# Autodesk Inventor assembly: khung
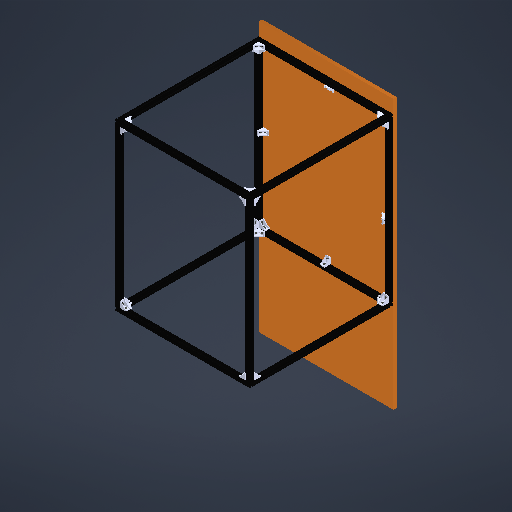
[picture p0: Inventor's stored thumbnail of the model, 512x512]
Saved by Autodesk Inventor 2027.1 (Build 311270010, 270A)
## iProperties
Created: 2026-08-09
Part Number: khung
Document SubType Name: Assembly
Designer: MSI
Author: MSI
## Documents named in this file (6)
- C:\Users\MSI\Documents\MECHATRONICS\Tot_nghiep\Do_an_Delta.Robot_Dang_Rui_Bi\Thiết kế\Delta Part\khung.iam
- C:\Users\MSI\Documents\MECHATRONICS\Tot_nghiep\Do_an_Delta.Robot_Dang_Rui_Bi\Thiết kế\Delta Part\tấm gỗ.ipt
- C:\Users\MSI\Documents\MECHATRONICS\Tot_nghiep\Do_an_Delta.Robot_Dang_Rui_Bi\Thiết kế\Delta Part\nhôm định hình 20x20_600.ipt
- C:\Users\MSI\Documents\MECHATRONICS\Tot_nghiep\Do_an_Delta.Robot_Dang_Rui_Bi\Thiết kế\Delta Part\nhôm định hình 20x20_700.ipt
- C:\Users\MSI\Documents\MECHATRONICS\Tot_nghiep\Do_an_Delta.Robot_Dang_Rui_Bi\Thiết kế\Delta Part\ke góc.ipt
- C:\Users\MSI\Documents\Inventor\Content Center Files\R2027\en-US\ISO 7380-1\ISO 7380-1 - M5 x 8.ipt
## Components (100 placed, 5 different names)
1. tấm gỗ:1 — Flush:1, Mate:1, Flush:2, Mate:3, Flush:4, Mate:5, Flush:5, Mate:66, Mate:67, Mate:68, Mate:69
2. nhôm định hình 20x20_600:1 — Flush:1, Mate:1, Mate:2, Flush:3, Mate:4, Mate:10, Flush:10, Flush:11, Mate:11, Flush:12, Flush:13, Mate:21, Mate:22, Flush:24, Mate:27, Mate:30, Flush:28, Mate:71
3. nhôm định hình 20x20_700:1 — Mate:2, Flush:2, Flush:3, Mate:7, Mate:19, Mate:20, Flush:22, Flush:23, Mate:32, Flush:29, Mate:36, Mate:70
4. nhôm định hình 20x20_700:2 — Mate:3, Flush:4, Mate:4, Mate:6, Mate:8, Flush:6, Mate:23, Mate:25, Mate:28, Mate:38, Mate:73
5. nhôm định hình 20x20_600:2 — Mate:5, Mate:6, Mate:7, Flush:5, Flush:7, Mate:9, Flush:8, Flush:9, Mate:18, Mate:24, Flush:25, Mate:35, Mate:40, Mate:72
6. nhôm định hình 20x20_600:3 — Mate:10, Flush:10, Flush:11, Mate:13, Mate:31, Mate:33, Mate:54, Mate:56, Flush:41
7. nhôm định hình 20x20_600:4 — Mate:11, Flush:12, Flush:13, Mate:12, Flush:14, Flush:15, Mate:14, Mate:26, Flush:26, Mate:29, Flush:27, Mate:50, Mate:52
8. nhôm định hình 20x20_600:5 — Mate:9, Flush:8, Flush:9, Mate:15, Flush:17, Mate:34, Flush:30, Mate:37, Flush:31, Mate:43, Flush:34, Mate:44
9. nhôm định hình 20x20_600:6 — Mate:8, Flush:6, Flush:7, Flush:16, Mate:39, Flush:32, Mate:41, Flush:33, Mate:46, Flush:36, Mate:48
10. nhôm định hình 20x20_600:7 — Mate:15, Flush:16, Flush:17, Mate:16, Flush:19, Mate:17, Mate:42, Mate:47, Mate:59, Flush:42, Mate:64, Flush:45
11. nhôm định hình 20x20_600:8 — Mate:12, Mate:13, Flush:14, Flush:15, Mate:14, Flush:18, Flush:20, Flush:21, Mate:53, Flush:39, Mate:55, Flush:40, Mate:61, Flush:43, Mate:62
12. nhôm định hình 20x20_700:3 — Mate:16, Flush:18, Flush:19, Mate:45, Flush:35, Mate:57, Mate:58, Mate:60
13. nhôm định hình 20x20_700:4 — Mate:17, Flush:20, Flush:21, Mate:49, Flush:37, Mate:51, Flush:38, Mate:63, Flush:44, Mate:65
14. ke góc:1 — Mate:28, Mate:29, Flush:27, Insert:23, Insert:24
15. ke góc:2 — Mate:32, Mate:33, Flush:29, Insert:31, Insert:32
16. ke góc:3 — Mate:38, Mate:39, Flush:32, Insert:5, Insert:6, Insert:9
17. ke góc:4 — Mate:36, Mate:37, Flush:31, Insert:12, Insert:13
18. ke góc:5 — Mate:34, Mate:35, Flush:30, Insert:16, Insert:17
19. ke góc:6 — Mate:26, Mate:27, Flush:26, Insert:21, Insert:22
20. ke góc:7 — Mate:24, Mate:25, Flush:25, Insert:1, Insert:2, Insert:3, Insert:4
21. ke góc:8 — Mate:18, Mate:19, Flush:23, Insert:14, Insert:15
22. ke góc:9 — Mate:22, Flush:24, Mate:23, Insert:25, Insert:26
23. ke góc:10 — Mate:20, Mate:21, Flush:22, Insert:29, Insert:30
24. ke góc:11 — Mate:30, Mate:31, Flush:28, Insert:33, Insert:34
25. ke góc:12 — Mate:46, Mate:47, Flush:36, Insert:39, Insert:40
26. ke góc:13 — Mate:58, Mate:59, Flush:42, Insert:54, Insert:55
27. ke góc:14 — Mate:56, Mate:57, Flush:41, Insert:47, Insert:52
28. ke góc:15 — Mate:52, Mate:53, Flush:39, Insert:41, Insert:42
29. ke góc:16 — Mate:48, Mate:49, Flush:37, Insert:35, Insert:37
30. ke góc:17 — Mate:50, Mate:51, Flush:38, Insert:45, Insert:46
31. ke góc:18 — Mate:44, Mate:45, Flush:35, Insert:57, Insert:58
32. ke góc:19 — Mate:42, Mate:43, Flush:34, Insert:53, Insert:56
33. ke góc:20 — Mate:54, Mate:55, Flush:40, Insert:50, Insert:51
34. ke góc:21 — Mate:40, Mate:41, Flush:33, Insert:7, Insert:8
35. ke góc:22 — Mate:60, Mate:61, Flush:43, Insert:48, Insert:49
36. ke góc:23 — Mate:62, Mate:63, Flush:44, Insert:43, Insert:44
37. ke góc:24 — Mate:64, Mate:65, Flush:45, Insert:36, Insert:38
38. ke góc:25 — Mate:66, Mate:70, Mate:74, Mate:75, Insert:18
39. ke góc:26 — Mate:69, Mate:72, Insert:10, Insert:11
40. ke góc:27 — Mate:68, Mate:71, Insert:27, Insert:28
41. ke góc:28 — Mate:67, Mate:73, Insert:19, Insert:20
42. ISO 7380-1 M5 x 8:1 — Insert:1
43. ISO 7380-1 M5 x 8:2 — Insert:2
44. ISO 7380-1 M5 x 8:3 — Insert:3
45. ISO 7380-1 M5 x 8:4 — Insert:4
46. ISO 7380-1 M5 x 8:5 — Insert:5
47. ISO 7380-1 M5 x 8:6 — Insert:6
48. ISO 7380-1 M5 x 8:7 — Insert:7
49. ISO 7380-1 M5 x 8:8 — Insert:8
50. ISO 7380-1 M5 x 8:9 — Insert:9
51. ISO 7380-1 M5 x 8:10 — Insert:10
52. ISO 7380-1 M5 x 8:11 — Insert:11
53. ISO 7380-1 M5 x 8:12 — Insert:12
54. ISO 7380-1 M5 x 8:13 — Insert:13
55. ISO 7380-1 M5 x 8:14 — Insert:14
56. ISO 7380-1 M5 x 8:15 — Insert:15
57. ISO 7380-1 M5 x 8:16 — Insert:16
58. ISO 7380-1 M5 x 8:17 — Insert:17
59. ISO 7380-1 M5 x 8:18 — Mate:74, Mate:75
60. ISO 7380-1 M5 x 8:19 — Insert:18
61. ISO 7380-1 M5 x 8:20 — Insert:19
62. ISO 7380-1 M5 x 8:21 — Insert:20
63. ISO 7380-1 M5 x 8:22 — Insert:21
64. ISO 7380-1 M5 x 8:23 — Insert:22
65. ISO 7380-1 M5 x 8:24 — Insert:23
66. ISO 7380-1 M5 x 8:25 — Insert:24
67. ISO 7380-1 M5 x 8:26 — Insert:25
68. ISO 7380-1 M5 x 8:27 — Insert:26
69. ISO 7380-1 M5 x 8:28 — Insert:27
70. ISO 7380-1 M5 x 8:29 — Insert:28
71. ISO 7380-1 M5 x 8:30 — Insert:29
72. ISO 7380-1 M5 x 8:31 — Insert:30
73. ISO 7380-1 M5 x 8:32 — Insert:31
74. ISO 7380-1 M5 x 8:33 — Insert:32
75. ISO 7380-1 M5 x 8:34 — Insert:33
76. ISO 7380-1 M5 x 8:35 — Insert:34
77. ISO 7380-1 M5 x 8:36 — Insert:35
78. ISO 7380-1 M5 x 8:37 — Insert:36
79. ISO 7380-1 M5 x 8:38 — Insert:37
80. ISO 7380-1 M5 x 8:39 — Insert:38
81. ISO 7380-1 M5 x 8:40 — Insert:39
82. ISO 7380-1 M5 x 8:41 — Insert:40
83. ISO 7380-1 M5 x 8:42 — Insert:41
84. ISO 7380-1 M5 x 8:43 — Insert:42
85. ISO 7380-1 M5 x 8:44 — Insert:43
86. ISO 7380-1 M5 x 8:45 — Insert:44
87. ISO 7380-1 M5 x 8:46 — Insert:45
88. ISO 7380-1 M5 x 8:47 — Insert:46
89. ISO 7380-1 M5 x 8:48 — Insert:47
90. ISO 7380-1 M5 x 8:49 — Insert:48
91. ISO 7380-1 M5 x 8:50 — Insert:49
92. ISO 7380-1 M5 x 8:51 — Insert:50
93. ISO 7380-1 M5 x 8:52 — Insert:51
94. ISO 7380-1 M5 x 8:53 — Insert:52
95. ISO 7380-1 M5 x 8:54 — Insert:53
96. ISO 7380-1 M5 x 8:55 — Insert:54
97. ISO 7380-1 M5 x 8:56 — Insert:55
98. ISO 7380-1 M5 x 8:57 — Insert:56
99. ISO 7380-1 M5 x 8:58 — Insert:57
100. ISO 7380-1 M5 x 8:59 — Insert:58
## Relationships (178: Mate 75, Insert 58, Flush 45)
- Flush:1: tấm gỗ:1 ↔ nhôm định hình 20x20_600:1
- Mate:1: tấm gỗ:1 ↔ nhôm định hình 20x20_600:1
- Mate:2: nhôm định hình 20x20_600:1 ↔ nhôm định hình 20x20_700:1
- Flush:2: tấm gỗ:1 ↔ nhôm định hình 20x20_700:1
- Flush:3: nhôm định hình 20x20_600:1 ↔ nhôm định hình 20x20_700:1
- Mate:3: tấm gỗ:1 ↔ nhôm định hình 20x20_700:2
- Flush:4: tấm gỗ:1 ↔ nhôm định hình 20x20_700:2
- Mate:4: nhôm định hình 20x20_600:1 ↔ nhôm định hình 20x20_700:2
- Mate:5: tấm gỗ:1 ↔ nhôm định hình 20x20_600:2
- Mate:6: nhôm định hình 20x20_700:2 ↔ nhôm định hình 20x20_600:2
- Mate:7: nhôm định hình 20x20_700:1 ↔ nhôm định hình 20x20_600:2
- Flush:5: tấm gỗ:1 ↔ nhôm định hình 20x20_600:2
- Mate:8: nhôm định hình 20x20_700:2 ↔ nhôm định hình 20x20_600:6
- Flush:6: nhôm định hình 20x20_700:2 ↔ nhôm định hình 20x20_600:6
- Flush:7: nhôm định hình 20x20_600:2 ↔ nhôm định hình 20x20_600:6
- Mate:9: nhôm định hình 20x20_600:2 ↔ nhôm định hình 20x20_600:5
- Flush:8: nhôm định hình 20x20_600:2 ↔ nhôm định hình 20x20_600:5
- Flush:9: nhôm định hình 20x20_600:2 ↔ nhôm định hình 20x20_600:5
- Mate:10: nhôm định hình 20x20_600:1 ↔ nhôm định hình 20x20_600:3
- Flush:10: nhôm định hình 20x20_600:1 ↔ nhôm định hình 20x20_600:3
- Flush:11: nhôm định hình 20x20_600:1 ↔ nhôm định hình 20x20_600:3
- Mate:11: nhôm định hình 20x20_600:1 ↔ nhôm định hình 20x20_600:4
- Flush:12: nhôm định hình 20x20_600:1 ↔ nhôm định hình 20x20_600:4
- Flush:13: nhôm định hình 20x20_600:1 ↔ nhôm định hình 20x20_600:4
- Mate:12: nhôm định hình 20x20_600:4 ↔ nhôm định hình 20x20_600:8
- Mate:13: nhôm định hình 20x20_600:3 ↔ nhôm định hình 20x20_600:8
- Flush:14: nhôm định hình 20x20_600:4 ↔ nhôm định hình 20x20_600:8
- Flush:15: nhôm định hình 20x20_600:4 ↔ nhôm định hình 20x20_600:8
- Mate:14: nhôm định hình 20x20_600:4 ↔ nhôm định hình 20x20_600:8
- Mate:15: nhôm định hình 20x20_600:5 ↔ nhôm định hình 20x20_600:7
- Flush:16: nhôm định hình 20x20_600:6 ↔ nhôm định hình 20x20_600:7
- Flush:17: nhôm định hình 20x20_600:5 ↔ nhôm định hình 20x20_600:7
- Mate:16: nhôm định hình 20x20_600:7 ↔ nhôm định hình 20x20_700:3
- Flush:18: nhôm định hình 20x20_600:8 ↔ nhôm định hình 20x20_700:3
- Flush:19: nhôm định hình 20x20_600:7 ↔ nhôm định hình 20x20_700:3
- Mate:17: nhôm định hình 20x20_600:7 ↔ nhôm định hình 20x20_700:4
- Flush:20: nhôm định hình 20x20_600:8 ↔ nhôm định hình 20x20_700:4
- Flush:21: nhôm định hình 20x20_600:8 ↔ nhôm định hình 20x20_700:4
- Mate:18: nhôm định hình 20x20_600:2 ↔ ke góc:8
- Mate:19: nhôm định hình 20x20_700:1 ↔ ke góc:8
- Mate:20: nhôm định hình 20x20_700:1 ↔ ke góc:10
- Mate:21: nhôm định hình 20x20_600:1 ↔ ke góc:10
- Flush:22: nhôm định hình 20x20_700:1 ↔ ke góc:10
- Flush:23: nhôm định hình 20x20_700:1 ↔ ke góc:8
- Mate:22: nhôm định hình 20x20_600:1 ↔ ke góc:9
- Flush:24: nhôm định hình 20x20_600:1 ↔ ke góc:9
- Mate:23: nhôm định hình 20x20_700:2 ↔ ke góc:9
- Mate:24: nhôm định hình 20x20_600:2 ↔ ke góc:7
- Mate:25: nhôm định hình 20x20_700:2 ↔ ke góc:7
- Flush:25: nhôm định hình 20x20_600:2 ↔ ke góc:7
- Mate:26: nhôm định hình 20x20_600:4 ↔ ke góc:6
- Mate:27: nhôm định hình 20x20_600:1 ↔ ke góc:6
- Flush:26: nhôm định hình 20x20_600:4 ↔ ke góc:6
- Mate:28: nhôm định hình 20x20_700:2 ↔ ke góc:1
- Mate:29: nhôm định hình 20x20_600:4 ↔ ke góc:1
- Flush:27: nhôm định hình 20x20_600:4 ↔ ke góc:1
- Mate:30: nhôm định hình 20x20_600:1 ↔ ke góc:11
- Mate:31: nhôm định hình 20x20_600:3 ↔ ke góc:11
- Flush:28: nhôm định hình 20x20_600:1 ↔ ke góc:11
- Mate:32: nhôm định hình 20x20_700:1 ↔ ke góc:2
- Mate:33: nhôm định hình 20x20_600:3 ↔ ke góc:2
- Flush:29: nhôm định hình 20x20_700:1 ↔ ke góc:2
- Mate:34: nhôm định hình 20x20_600:5 ↔ ke góc:5
- Mate:35: nhôm định hình 20x20_600:2 ↔ ke góc:5
- Flush:30: nhôm định hình 20x20_600:5 ↔ ke góc:5
- Mate:36: nhôm định hình 20x20_700:1 ↔ ke góc:4
- Mate:37: nhôm định hình 20x20_600:5 ↔ ke góc:4
- Flush:31: nhôm định hình 20x20_600:5 ↔ ke góc:4
- Mate:38: nhôm định hình 20x20_700:2 ↔ ke góc:3
- Mate:39: nhôm định hình 20x20_600:6 ↔ ke góc:3
- Flush:32: nhôm định hình 20x20_600:6 ↔ ke góc:3
- Mate:40: nhôm định hình 20x20_600:2 ↔ ke góc:21
- Mate:41: nhôm định hình 20x20_600:6 ↔ ke góc:21
- Flush:33: nhôm định hình 20x20_600:6 ↔ ke góc:21
- Mate:42: nhôm định hình 20x20_600:7 ↔ ke góc:19
- Mate:43: nhôm định hình 20x20_600:5 ↔ ke góc:19
- Flush:34: nhôm định hình 20x20_600:5 ↔ ke góc:19
- Mate:44: nhôm định hình 20x20_600:5 ↔ ke góc:18
- Mate:45: nhôm định hình 20x20_700:3 ↔ ke góc:18
- Flush:35: nhôm định hình 20x20_700:3 ↔ ke góc:18
- Mate:46: nhôm định hình 20x20_600:6 ↔ ke góc:12
- Mate:47: nhôm định hình 20x20_600:7 ↔ ke góc:12
- Flush:36: nhôm định hình 20x20_600:6 ↔ ke góc:12
- Mate:48: nhôm định hình 20x20_600:6 ↔ ke góc:16
- Mate:49: nhôm định hình 20x20_700:4 ↔ ke góc:16
- Flush:37: nhôm định hình 20x20_700:4 ↔ ke góc:16
- Mate:50: nhôm định hình 20x20_600:4 ↔ ke góc:17
- Mate:51: nhôm định hình 20x20_700:4 ↔ ke góc:17
- Flush:38: nhôm định hình 20x20_700:4 ↔ ke góc:17
- Mate:52: nhôm định hình 20x20_600:4 ↔ ke góc:15
- Mate:53: nhôm định hình 20x20_600:8 ↔ ke góc:15
- Flush:39: nhôm định hình 20x20_600:8 ↔ ke góc:15
- Mate:54: nhôm định hình 20x20_600:3 ↔ ke góc:20
- Mate:55: nhôm định hình 20x20_600:8 ↔ ke góc:20
- Flush:40: nhôm định hình 20x20_600:8 ↔ ke góc:20
- Mate:56: nhôm định hình 20x20_600:3 ↔ ke góc:14
- Mate:57: nhôm định hình 20x20_700:3 ↔ ke góc:14
- Flush:41: nhôm định hình 20x20_600:3 ↔ ke góc:14
- Mate:58: nhôm định hình 20x20_700:3 ↔ ke góc:13
- Mate:59: nhôm định hình 20x20_600:7 ↔ ke góc:13
- Flush:42: nhôm định hình 20x20_600:7 ↔ ke góc:13
- Mate:60: nhôm định hình 20x20_700:3 ↔ ke góc:22
- Mate:61: nhôm định hình 20x20_600:8 ↔ ke góc:22
- Flush:43: nhôm định hình 20x20_600:8 ↔ ke góc:22
- Mate:62: nhôm định hình 20x20_600:8 ↔ ke góc:23
- Mate:63: nhôm định hình 20x20_700:4 ↔ ke góc:23
- Flush:44: nhôm định hình 20x20_700:4 ↔ ke góc:23
- Mate:64: nhôm định hình 20x20_600:7 ↔ ke góc:24
- Mate:65: nhôm định hình 20x20_700:4 ↔ ke góc:24
- Flush:45: nhôm định hình 20x20_600:7 ↔ ke góc:24
- Mate:66: tấm gỗ:1 ↔ ke góc:25
- Mate:67: tấm gỗ:1 ↔ ke góc:28
- Mate:68: tấm gỗ:1 ↔ ke góc:27
- Mate:69: tấm gỗ:1 ↔ ke góc:26
- Mate:70: nhôm định hình 20x20_700:1 ↔ ke góc:25
- Mate:71: nhôm định hình 20x20_600:1 ↔ ke góc:27
- Mate:72: nhôm định hình 20x20_600:2 ↔ ke góc:26
- Mate:73: nhôm định hình 20x20_700:2 ↔ ke góc:28
- Insert:1: ke góc:7 ↔ ISO 7380-1 M5 x 8:1
- Insert:2: ke góc:7 ↔ ISO 7380-1 M5 x 8:2
- Insert:3: ke góc:7 ↔ ISO 7380-1 M5 x 8:3
- Insert:4: ke góc:7 ↔ ISO 7380-1 M5 x 8:4
- Insert:5: ke góc:3 ↔ ISO 7380-1 M5 x 8:5
- Insert:6: ke góc:3 ↔ ISO 7380-1 M5 x 8:6
- Insert:7: ke góc:21 ↔ ISO 7380-1 M5 x 8:7
- Insert:8: ke góc:21 ↔ ISO 7380-1 M5 x 8:8
- Insert:9: ke góc:3 ↔ ISO 7380-1 M5 x 8:9
- Insert:10: ke góc:26 ↔ ISO 7380-1 M5 x 8:10
- Insert:11: ke góc:26 ↔ ISO 7380-1 M5 x 8:11
- Insert:12: ke góc:4 ↔ ISO 7380-1 M5 x 8:12
- Insert:13: ke góc:4 ↔ ISO 7380-1 M5 x 8:13
- Insert:14: ke góc:8 ↔ ISO 7380-1 M5 x 8:14
- Insert:15: ke góc:8 ↔ ISO 7380-1 M5 x 8:15
- Insert:16: ke góc:5 ↔ ISO 7380-1 M5 x 8:16
- Insert:17: ke góc:5 ↔ ISO 7380-1 M5 x 8:17
- Mate:74: ke góc:25 ↔ ISO 7380-1 M5 x 8:18
- Mate:75: ke góc:25 ↔ ISO 7380-1 M5 x 8:18
- Insert:18: ke góc:25 ↔ ISO 7380-1 M5 x 8:19
- Insert:19: ke góc:28 ↔ ISO 7380-1 M5 x 8:20
- Insert:20: ke góc:28 ↔ ISO 7380-1 M5 x 8:21
- Insert:21: ke góc:6 ↔ ISO 7380-1 M5 x 8:22
- Insert:22: ke góc:6 ↔ ISO 7380-1 M5 x 8:23
- Insert:23: ke góc:1 ↔ ISO 7380-1 M5 x 8:24
- Insert:24: ke góc:1 ↔ ISO 7380-1 M5 x 8:25
- Insert:25: ke góc:9 ↔ ISO 7380-1 M5 x 8:26
- Insert:26: ke góc:9 ↔ ISO 7380-1 M5 x 8:27
- Insert:27: ke góc:27 ↔ ISO 7380-1 M5 x 8:28
- Insert:28: ke góc:27 ↔ ISO 7380-1 M5 x 8:29
- Insert:29: ke góc:10 ↔ ISO 7380-1 M5 x 8:30
- Insert:30: ke góc:10 ↔ ISO 7380-1 M5 x 8:31
- Insert:31: ke góc:2 ↔ ISO 7380-1 M5 x 8:32
- Insert:32: ke góc:2 ↔ ISO 7380-1 M5 x 8:33
- Insert:33: ke góc:11 ↔ ISO 7380-1 M5 x 8:34
- Insert:34: ke góc:11 ↔ ISO 7380-1 M5 x 8:35
- Insert:35: ke góc:16 ↔ ISO 7380-1 M5 x 8:36
- Insert:36: ke góc:24 ↔ ISO 7380-1 M5 x 8:37
- Insert:37: ke góc:16 ↔ ISO 7380-1 M5 x 8:38
- Insert:38: ke góc:24 ↔ ISO 7380-1 M5 x 8:39
- Insert:39: ke góc:12 ↔ ISO 7380-1 M5 x 8:40
- Insert:40: ke góc:12 ↔ ISO 7380-1 M5 x 8:41
- Insert:41: ke góc:15 ↔ ISO 7380-1 M5 x 8:42
- Insert:42: ke góc:15 ↔ ISO 7380-1 M5 x 8:43
- Insert:43: ke góc:23 ↔ ISO 7380-1 M5 x 8:44
- Insert:44: ke góc:23 ↔ ISO 7380-1 M5 x 8:45
- Insert:45: ke góc:17 ↔ ISO 7380-1 M5 x 8:46
- Insert:46: ke góc:17 ↔ ISO 7380-1 M5 x 8:47
- Insert:47: ke góc:14 ↔ ISO 7380-1 M5 x 8:48
- Insert:48: ke góc:22 ↔ ISO 7380-1 M5 x 8:49
- Insert:49: ke góc:22 ↔ ISO 7380-1 M5 x 8:50
- Insert:50: ke góc:20 ↔ ISO 7380-1 M5 x 8:51
- Insert:51: ke góc:20 ↔ ISO 7380-1 M5 x 8:52
- Insert:52: ke góc:14 ↔ ISO 7380-1 M5 x 8:53
- Insert:53: ke góc:19 ↔ ISO 7380-1 M5 x 8:54
- Insert:54: ke góc:13 ↔ ISO 7380-1 M5 x 8:55
- Insert:55: ke góc:13 ↔ ISO 7380-1 M5 x 8:56
- Insert:56: ke góc:19 ↔ ISO 7380-1 M5 x 8:57
- Insert:57: ke góc:18 ↔ ISO 7380-1 M5 x 8:58
- Insert:58: ke góc:18 ↔ ISO 7380-1 M5 x 8:59
